# Autodesk Inventor assembly: biotrap-base-sensor
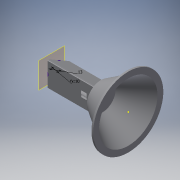
[picture p0: Inventor's stored thumbnail of the model, 180x180]
Saved by Autodesk Inventor 2017 (Build 210142000, 142)
## iProperties
Created: 2018-06-28
Part Number: biotrap-base-sensor
Document SubType Name: Assembly
Designer: 45027374
Author: 45027374
## Documents named in this file (3)
- C:\Users\45027374\cloudstor\Documents\3Dprints\fruitfly-counter\biotrap-base-sensor.iam
- C:\Users\45027374\cloudstor\Documents\3Dprints\fruitfly-counter\base-biotrap.ipt
- C:\Users\45027374\cloudstor\Documents\3Dprints\fruitfly-counter\counter-adapter-USA-trap-v4.ipt
## Components (2 placed, 2 different names)
1. base-biotrap:1 — Mate:1, Mate:2, Mate:3, Mate:7
2. counter-adapter-USA-trap-v4:1 — Mate:4, Mate:6, Mate:7
## Relationships (6: Mate 6)
- Mate:1: base-biotrap:1
- Mate:2: base-biotrap:1
- Mate:3: base-biotrap:1
- Mate:4: counter-adapter-USA-trap-v4:1
- Mate:6: counter-adapter-USA-trap-v4:1
- Mate:7: base-biotrap:1 ↔ counter-adapter-USA-trap-v4:1
